# Autodesk Inventor assembly: Assembly1
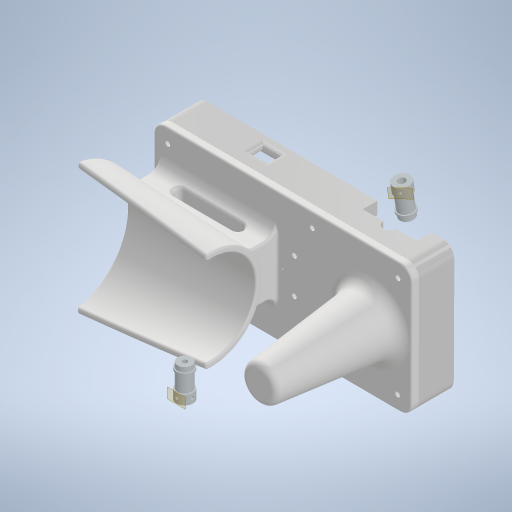
[picture p0: Inventor's stored thumbnail of the model, 512x512]
Saved by Autodesk Inventor 2024 (Build 280153000, 153)
## iProperties
Created: 2023-07-30
Part Number: Assembly1
Document SubType Name: Assembly
Designer: Pintu
Author: Pintu
## Documents named in this file (6)
- D:\CMC\my_inventor\ArmBo_v2\Assembly1.iam
- D:\CMC\my_inventor\ArmBo_v2\Bottom_chassis.ipt
- D:\CMC\my_inventor\ArmBo_v2\hand_rest.ipt
- D:\CMC\my_inventor\ArmBo_v2\imu_holder.ipt
- D:\CMC\my_inventor\ArmBo_v2\support\ShaftConnector.ipt
- D:\CMC\my_inventor\ArmBo_v2\ORANGE_ENCODER\ORANGE_ENCODER_600PPR v1.ipt
## Components (8 placed, 5 different names)
1. Bottom_chassis:1 — Mate:1, Mate:2, Mate:4, Mate:5, Mate:6, Mate:7, Mate:8, Mate:9
2. hand_rest:1 — Mate:1, Mate:2, Mate:3
3. imu_holder:1 — Mate:3
4. ShaftConnector:1
5. ShaftConnector:2
6. ORANGE_ENCODER_600PPR v1:1 — Mate:4, Mate:5
7. ORANGE_ENCODER_600PPR v1:2 — Mate:8, Mate:9
8. ORANGE_ENCODER_600PPR v1:3 — Mate:6, Mate:7
## Relationships (9: Mate 9)
- Mate:1: Bottom_chassis:1 ↔ hand_rest:1
- Mate:2: Bottom_chassis:1 ↔ hand_rest:1
- Mate:3: hand_rest:1 ↔ imu_holder:1
- Mate:4: Bottom_chassis:1 ↔ ORANGE_ENCODER_600PPR v1:1
- Mate:5: Bottom_chassis:1 ↔ ORANGE_ENCODER_600PPR v1:1
- Mate:6: Bottom_chassis:1 ↔ ORANGE_ENCODER_600PPR v1:3
- Mate:7: Bottom_chassis:1 ↔ ORANGE_ENCODER_600PPR v1:3
- Mate:8: Bottom_chassis:1 ↔ ORANGE_ENCODER_600PPR v1:2
- Mate:9: Bottom_chassis:1 ↔ ORANGE_ENCODER_600PPR v1:2
